# Autodesk Inventor assembly: Сборка_новая
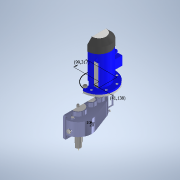
[picture p0: Inventor's stored thumbnail of the model, 180x180]
Saved by Autodesk Inventor 2021 (Build 250183000, 183)
## iProperties
Created: 2023-04-22
Part Number: Сборка_новая
Document SubType Name: Assembly
Designer: gdevc
Mass: 20918.9 g
Surface Area: 13939.4 cm^2
Volume: 12393.5 cm^3
Density: 1.6879 g/cm^3
Author: gdevc
## Documents named in this file (29)
- C:\Users\gdevc\OneDrive\Рабочий стол\Курсач\DetaliMashine\Новая папка\Сборка_новая.iam
- C:\Users\gdevc\OneDrive\Рабочий стол\Курсач\DetaliMashine\Новая папка\Корпус.v.2.0.iam
- C:\Users\gdevc\OneDrive\Рабочий стол\Курсач\DetaliMashine\Новая папка\Вал_тихоходный.ipt
- C:\Users\gdevc\OneDrive\Рабочий стол\Курсач\DetaliMashine\Новая папка\Чертежи\Подшипник 7210A ГОСТ 27365-87.ipt
- C:\Users\gdevc\OneDrive\Рабочий стол\Курсач\DetaliMashine\Новая папка\Крышка тих_выход.ipt
- C:\Users\gdevc\OneDrive\Рабочий стол\Курсач\DetaliMashine\Новая папка\Вал_промежуточный.ipt
- C:\Users\gdevc\OneDrive\Рабочий стол\Курсач\DetaliMashine\Новая папка\Подшипник 7205A ГОСТ 27365-8v.1.ipt
- C:\Users\gdevc\OneDrive\Рабочий стол\Курсач\DetaliMashine\Новая папка\Крышка_пром.ipt
- C:\Users\gdevc\OneDrive\Рабочий стол\Курсач\DetaliMashine\Новая папка\Колесо быстроходное.ipt
- C:\Users\gdevc\OneDrive\Рабочий стол\Курсач\DetaliMashine\Новая папка\Валл быстроходный.ipt
- C:\Users\gdevc\OneDrive\Рабочий стол\Курсач\DetaliMashine\Новая папка\Крышка_быстроходного.ipt
- C:\Users\gdevc\OneDrive\Рабочий стол\Курсач\DetaliMashine\Новая папка\Манжет 2-50x65x8 ГОСТ 8752-79.ipt
- C:\Users\gdevc\OneDrive\Рабочий стол\Курсач\DetaliMashine\Новая папка\Манжет 1-30x47x7 ГОСТ 8752-79.ipt
- C:\Users\gdevc\Downloads\Telegram Desktop\АИР100L IM2081 (2,4,6,8 пол)....ipt
- C:\Users\gdevc\OneDrive\Рабочий стол\Курсач\DetaliMashine\Новая папка\Резина конец.ipt
- C:\Users\gdevc\OneDrive\Рабочий стол\Курсач\DetaliMashine\Новая папка\Промежуточное колесо резина.ipt
- C:\Users\gdevc\OneDrive\Документы\Inventor\Content Center Files\R2021\ru-RU\GOST 5915-70\Гайка M16-6H ГОСТ 5915-70(1).ipt
- C:\Users\gdevc\OneDrive\Рабочий стол\Курсач\DetaliMashine\Новая папка\Слив_масла.ipt
- C:\Users\gdevc\Downloads\prokladka_GOST_15180-86.ipt
- C:\Users\gdevc\OneDrive\Рабочий стол\Курсач\DetaliMashine\Новая папка\Шуп масло.ipt
- C:\Users\gdevc\OneDrive\Рабочий стол\Курсач\DetaliMashine\Новая папка\Манжет 2-55x72x8 ГОСТ 8752-79.ipt
- C:\Users\gdevc\OneDrive\Рабочий стол\Курсач\DetaliMashine\Новая папка\Регулировка.ipt
- C:\Users\gdevc\OneDrive\Рабочий стол\Курсач\DetaliMashine\Новая папка\Крышка_пром_новая.ipt
- C:\Users\gdevc\OneDrive\Рабочий стол\Курсач\DetaliMashine\Новая папка\Винт M10-6gx25 ГОСТ 1491-80.ipt
- C:\Users\gdevc\OneDrive\Рабочий стол\Курсач\DetaliMashine\Новая папка\Копия Копия гайки M10x1-6H ГОСТ 5915-70.ipt
- C:\Users\gdevc\OneDrive\Рабочий стол\Курсач\DetaliMashine\Новая папка\Регулировка-тихая.ipt
- C:\Users\gdevc\OneDrive\Рабочий стол\Курсач\DetaliMashine\Новая папка\Крышка тих.ipt
- C:\Users\gdevc\OneDrive\Рабочий стол\Курсач\DetaliMashine\Новая папка\Винт M10-6gx20 ГОСТ 1491-80.ipt
- C:\Users\gdevc\OneDrive\Рабочий стол\Курсач\DetaliMashine\Новая папка\Валл_резина.ipt
## Components (31 placed, 28 different names)
1. Корпус.v.2.0:1 [sub-assembly] — Совмещение:1, Угол:1, Угол:2, Угол:3, Совмещение:7, Совмещение:10, Совмещение:11, Угол:4, Угол:5, Совмещение:19, Совмещение:22, Совмещение:24, Совмещение:25, Угол:6, Угол:7, Угол:9, Совмещение:37, Совмещение:38, Совмещение:41, Угол:10, Совмещение:42, Совмещение:43, Угол:11, Совмещение:56, Совмещение:57, Заподлицо:4, Угол:13, Угол:14, Совмещение:63, Заподлицо:5
2. Вал_тихоходный:1 — Совмещение:1, Угол:1, Совмещение:2, Совмещение:3, Совмещение:4, Совмещение:5, Совмещение:6, Заподлицо:1, Совмещение:26, Совмещение:32, Совмещение:44, Совмещение:54, Совмещение:59, Совмещение:60
3. Подшипник 7210A ГОСТ 27365-87:1 — Совмещение:2, Совмещение:4, Угол:2
4. Подшипник 7210A ГОСТ 27365-87:2 — Совмещение:3, Совмещение:5, Угол:3, Совмещение:55
5. Крышка тих_выход:1 — Совмещение:6, Совмещение:7, Совмещение:27, Совмещение:45
6. Вал_промежуточный:1 — Совмещение:10, Заподлицо:1, Совмещение:13, Совмещение:14, Совмещение:15, Совмещение:17, Совмещение:20, Совмещение:46, Совмещение:47
7. Подшипник 7205A ГОСТ 27365-8v.1:1 — Совмещение:14, Совмещение:15, Угол:4, Совмещение:58
8. Подшипник 7205A ГОСТ 27365-8v.1:2 — Совмещение:11, Совмещение:13, Угол:5, Совмещение:52
9. Крышка_пром:2 — Совмещение:17, Совмещение:19, Совмещение:58
10. Колесо быстроходное:1 — Совмещение:20, Заподлицо:2
11. Валл быстроходный:1 — Совмещение:22, Совмещение:23, Совмещение:25, Заподлицо:2, Угол:6, Совмещение:28, Совмещение:30
12. Крышка_быстроходного:1 — Совмещение:23, Совмещение:24, Совмещение:29, Совмещение:31, Угол:8
13. Манжет 2-50x65x8 ГОСТ 8752-79:1 — Совмещение:26, Совмещение:27
14. Манжет 1-30x47x7 ГОСТ 8752-79:1 — Совмещение:28, Совмещение:29
15. АИР100L IM2081 (2,4,6,8 пол)...:1 — Угол:7, Совмещение:30, Совмещение:31, Угол:8, Совмещение:35, Совмещение:36
16. Резина конец:1 — Совмещение:64, Совмещение:65
17. Промежуточное колесо резина:1 — Совмещение:32
18. Гайка ГОСТ 5915-70 M16:1 — Совмещение:35, Совмещение:36, Угол:9, Совмещение:37
19. Слив_масла:1 — Совмещение:38, Совмещение:39, Совмещение:40, Угол:10
20. prokladka_GOST_15180-86:1 — Совмещение:39, Совмещение:40, Совмещение:41
21. Шуп масло:1 — Совмещение:42, Совмещение:43
22. Манжет 2-55x72x8 ГОСТ 8752-79:1 — Совмещение:44, Совмещение:45
23. Регулировка:1 — Совмещение:46, Совмещение:51, Совмещение:52
24. Крышка_пром_новая:1 — Совмещение:47, Совмещение:49, Совмещение:53, Заподлицо:4
25. Винт M10-6gx25 ГОСТ 1491-80:1 — Совмещение:49, Совмещение:50, Совмещение:51, Угол:11, Угол:12
26. Копия Копия гайки M10x1-6H ГОСТ 5915-70:1 — Совмещение:50, Угол:12, Совмещение:53
27. Регулировка-тихая:1 — Совмещение:54, Совмещение:55, Совмещение:61
28. Крышка тих:1 — Совмещение:56, Совмещение:57, Совмещение:62
29. Винт M10-6gx20 ГОСТ 1491-80:1 — Совмещение:59, Угол:13, Совмещение:61
30. Копия Копия гайки M10x1-6H ГОСТ 5915-70:2 — Совмещение:60, Совмещение:62, Угол:14
31. Валл_резина:1 — Совмещение:63, Заподлицо:5, Совмещение:64, Совмещение:65
## Relationships (74: Mate 56, Angle 14, Flush 4)
- Совмещение:1 [Mate]: Корпус.v.2.0:1 ↔ Вал_тихоходный:1
- Угол:1 [Angle] (180 deg): Корпус.v.2.0:1 ↔ Вал_тихоходный:1
- Совмещение:2 [Mate]: Вал_тихоходный:1 ↔ Подшипник 7210A ГОСТ 27365-87:1
- Совмещение:3 [Mate]: Вал_тихоходный:1 ↔ Подшипник 7210A ГОСТ 27365-87:2
- Совмещение:4 [Mate]: Вал_тихоходный:1 ↔ Подшипник 7210A ГОСТ 27365-87:1
- Угол:2 [Angle] (180 deg): Корпус.v.2.0:1 ↔ Подшипник 7210A ГОСТ 27365-87:1
- Совмещение:5 [Mate]: Вал_тихоходный:1 ↔ Подшипник 7210A ГОСТ 27365-87:2
- Угол:3 [Angle] (0 deg): Корпус.v.2.0:1 ↔ Подшипник 7210A ГОСТ 27365-87:2
- Совмещение:6 [Mate]: Вал_тихоходный:1 ↔ Крышка тих_выход:1
- Совмещение:7 [Mate]: Корпус.v.2.0:1 ↔ Крышка тих_выход:1
- Совмещение:10 [Mate]: Корпус.v.2.0:1 ↔ Вал_промежуточный:1
- Совмещение:11 [Mate]: Корпус.v.2.0:1 ↔ Подшипник 7205A ГОСТ 27365-8v.1:2
- Заподлицо:1 [Flush] (-1.5 mm): Вал_тихоходный:1 ↔ Вал_промежуточный:1
- Совмещение:13 [Mate]: Вал_промежуточный:1 ↔ Подшипник 7205A ГОСТ 27365-8v.1:2
- Совмещение:14 [Mate]: Вал_промежуточный:1 ↔ Подшипник 7205A ГОСТ 27365-8v.1:1
- Совмещение:15 [Mate]: Вал_промежуточный:1 ↔ Подшипник 7205A ГОСТ 27365-8v.1:1
- Угол:4 [Angle] (0 deg): Корпус.v.2.0:1 ↔ Подшипник 7205A ГОСТ 27365-8v.1:1
- Угол:5 [Angle] (90 deg): Корпус.v.2.0:1 ↔ Подшипник 7205A ГОСТ 27365-8v.1:2
- Совмещение:17 [Mate]: Вал_промежуточный:1 ↔ Крышка_пром:2
- Совмещение:19 [Mate]: Корпус.v.2.0:1 ↔ Крышка_пром:2
- Совмещение:20 [Mate]: Вал_промежуточный:1 ↔ Колесо быстроходное:1
- Совмещение:22 [Mate]: Корпус.v.2.0:1 ↔ Валл быстроходный:1
- Совмещение:23 [Mate]: Валл быстроходный:1 ↔ Крышка_быстроходного:1
- Совмещение:24 [Mate]: Корпус.v.2.0:1 ↔ Крышка_быстроходного:1
- Совмещение:25 [Mate]: Корпус.v.2.0:1 ↔ Валл быстроходный:1
- Заподлицо:2 [Flush] (-1 mm): Колесо быстроходное:1 ↔ Валл быстроходный:1
- Угол:6 [Angle] (0 deg): Корпус.v.2.0:1 ↔ Валл быстроходный:1
- Совмещение:26 [Mate]: Вал_тихоходный:1 ↔ Манжет 2-50x65x8 ГОСТ 8752-79:1
- Совмещение:27 [Mate]: Крышка тих_выход:1 ↔ Манжет 2-50x65x8 ГОСТ 8752-79:1
- Совмещение:28 [Mate]: Валл быстроходный:1 ↔ Манжет 1-30x47x7 ГОСТ 8752-79:1
- Совмещение:29 [Mate]: Крышка_быстроходного:1 ↔ Манжет 1-30x47x7 ГОСТ 8752-79:1
- Угол:7 [Angle] (0 deg): Корпус.v.2.0:1 ↔ АИР100L IM2081 (2,4,6,8 пол)...:1
- Совмещение:30 [Mate]: Валл быстроходный:1 ↔ АИР100L IM2081 (2,4,6,8 пол)...:1
- Совмещение:31 [Mate]: Крышка_быстроходного:1 ↔ АИР100L IM2081 (2,4,6,8 пол)...:1
- Угол:8 [Angle] (0 deg): Крышка_быстроходного:1 ↔ АИР100L IM2081 (2,4,6,8 пол)...:1
- Совмещение:32 [Mate]: Вал_тихоходный:1 ↔ Промежуточное колесо резина:1
- Совмещение:35 [Mate] (3 mm): АИР100L IM2081 (2,4,6,8 пол)...:1 ↔ Гайка ГОСТ 5915-70 M16:1
- Совмещение:36 [Mate] (-107.5 mm): АИР100L IM2081 (2,4,6,8 пол)...:1 ↔ Гайка ГОСТ 5915-70 M16:1
- Угол:9 [Angle] (90 deg): Корпус.v.2.0:1 ↔ Гайка ГОСТ 5915-70 M16:1
- Совмещение:37 [Mate]: Корпус.v.2.0:1 ↔ Гайка ГОСТ 5915-70 M16:1
- Совмещение:38 [Mate]: Корпус.v.2.0:1 ↔ Слив_масла:1
- Совмещение:39 [Mate]: Слив_масла:1 ↔ prokladka_GOST_15180-86:1
- Совмещение:40 [Mate]: Слив_масла:1 ↔ prokladka_GOST_15180-86:1
- Совмещение:41 [Mate]: Корпус.v.2.0:1 ↔ prokladka_GOST_15180-86:1
- Угол:10 [Angle] (90 deg): Корпус.v.2.0:1 ↔ Слив_масла:1
- Совмещение:42 [Mate]: Корпус.v.2.0:1 ↔ Шуп масло:1
- Совмещение:43 [Mate]: Корпус.v.2.0:1 ↔ Шуп масло:1
- Совмещение:44 [Mate]: Вал_тихоходный:1 ↔ Манжет 2-55x72x8 ГОСТ 8752-79:1
- Совмещение:45 [Mate]: Крышка тих_выход:1 ↔ Манжет 2-55x72x8 ГОСТ 8752-79:1
- Совмещение:46 [Mate]: Вал_промежуточный:1 ↔ Регулировка:1
- Совмещение:47 [Mate]: Вал_промежуточный:1 ↔ Крышка_пром_новая:1
- Совмещение:49 [Mate]: Крышка_пром_новая:1 ↔ Винт M10-6gx25 ГОСТ 1491-80:1
- Совмещение:50 [Mate]: Винт M10-6gx25 ГОСТ 1491-80:1 ↔ Копия Копия гайки M10x1-6H ГОСТ 5915-70:1
- Совмещение:51 [Mate]: Регулировка:1 ↔ Винт M10-6gx25 ГОСТ 1491-80:1
- Совмещение:52 [Mate]: Подшипник 7205A ГОСТ 27365-8v.1:2 ↔ Регулировка:1
- Угол:11 [Angle] (0 deg): Корпус.v.2.0:1 ↔ Винт M10-6gx25 ГОСТ 1491-80:1
- Угол:12 [Angle] (0 deg): Винт M10-6gx25 ГОСТ 1491-80:1 ↔ Копия Копия гайки M10x1-6H ГОСТ 5915-70:1
- Совмещение:53 [Mate]: Крышка_пром_новая:1 ↔ Копия Копия гайки M10x1-6H ГОСТ 5915-70:1
- Совмещение:54 [Mate]: Вал_тихоходный:1 ↔ Регулировка-тихая:1
- Совмещение:55 [Mate]: Подшипник 7210A ГОСТ 27365-87:2 ↔ Регулировка-тихая:1
- Совмещение:56 [Mate]: Корпус.v.2.0:1 ↔ Крышка тих:1
- Совмещение:57 [Mate]: Корпус.v.2.0:1 ↔ Крышка тих:1
- Совмещение:58 [Mate]: Подшипник 7205A ГОСТ 27365-8v.1:1 ↔ Крышка_пром:2
- Заподлицо:4 [Flush]: Корпус.v.2.0:1 ↔ Крышка_пром_новая:1
- Совмещение:59 [Mate]: Вал_тихоходный:1 ↔ Винт M10-6gx20 ГОСТ 1491-80:1
- Угол:13 [Angle] (0 deg): Корпус.v.2.0:1 ↔ Винт M10-6gx20 ГОСТ 1491-80:1
- Совмещение:60 [Mate]: Вал_тихоходный:1 ↔ Копия Копия гайки M10x1-6H ГОСТ 5915-70:2
- Совмещение:61 [Mate]: Регулировка-тихая:1 ↔ Винт M10-6gx20 ГОСТ 1491-80:1
- Совмещение:62 [Mate]: Крышка тих:1 ↔ Копия Копия гайки M10x1-6H ГОСТ 5915-70:2
- Угол:14 [Angle] (0 deg): Корпус.v.2.0:1 ↔ Копия Копия гайки M10x1-6H ГОСТ 5915-70:2
- Совмещение:63 [Mate]: Корпус.v.2.0:1 ↔ Валл_резина:1
- Заподлицо:5 [Flush]: Корпус.v.2.0:1 ↔ Валл_резина:1
- Совмещение:64 [Mate]: Резина конец:1 ↔ Валл_резина:1
- Совмещение:65 [Mate]: Резина конец:1 ↔ Валл_резина:1
